# Autodesk Inventor assembly: mainflap_replace
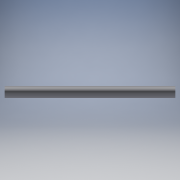
[picture p0: Inventor's stored thumbnail of the model, 180x180]
Saved by Autodesk Inventor 2018.2 (Build 222227000, 227)
## iProperties
Created: 2018-03-07
Part Number: mainflap_replace
Material: 一般
Document SubType Name: Assembly
Designer: ku_sk
Author: ku_sk
## Documents named in this file (2)
- C:\Users\ku_sk\Documents\Inventor\Aero\KS-15\Rr.wing\cradle\parts\mainflap_replace.iam
- C:\Users\ku_sk\Documents\Inventor\Aero\KS-15\Rr.wing\cradle\parts\main frap.ipt
## Components (1 placed, 1 different names)
1. main frap:1 — メイト:1, メイト:2, フラッシュ:1
## Relationships (3: Mate 2, Flush 1)
- メイト:1 [Mate]: main frap:1
- メイト:2 [Mate]: main frap:1
- フラッシュ:1 [Flush]: main frap:1
